# Autodesk Inventor assembly: Space
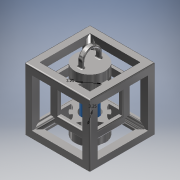
[picture p0: Inventor's stored thumbnail of the model, 180x180]
Saved by Autodesk Inventor 2019 (Build 230136000, 136)
## iProperties
Created: 2019-05-02
Part Number: Space
Document SubType Name: Assembly
Designer: Jorian Brusind
Author: Jorian Brusind
## Documents named in this file (4)
- C:\Users\Jorian Brusind\Documents\GitHub\PersonalProjects\Inventor Projects\Infinity\Space.iam
- C:\Users\Jorian Brusind\Documents\GitHub\PersonalProjects\Inventor Projects\Infinity\Inner.ipt
- C:\Users\Jorian Brusind\Documents\GitHub\PersonalProjects\Inventor Projects\Infinity\Blue.ipt
- C:\Users\Jorian Brusind\Documents\GitHub\PersonalProjects\Inventor Projects\Infinity\EndCap.ipt
## Components (4 placed, 3 different names)
1. Inner:1 — Mate:1, Mate:2, Mate:3, Mate:4, Flush:1
2. Blue:1 — Mate:1, Mate:5
3. EndCap:1 — Mate:3, Mate:4
4. EndCap:2 — Mate:2, Flush:1, Mate:5
## Relationships (6: Mate 5, Flush 1)
- Mate:1: Inner:1 ↔ Blue:1
- Mate:2: Inner:1 ↔ EndCap:2
- Mate:3: Inner:1 ↔ EndCap:1
- Mate:4: Inner:1 ↔ EndCap:1
- Flush:1: Inner:1 ↔ EndCap:2
- Mate:5 (-1 mm): Blue:1 ↔ EndCap:2
